# Autodesk Inventor assembly: Electronics V2
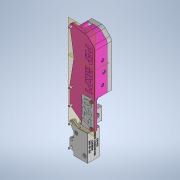
[picture p0: Inventor's stored thumbnail of the model, 180x180]
Saved by Autodesk Inventor 2020.3 (Build 243373010, 373A)
## iProperties
Created: 2019-12-13
Part Number: Electronics V2
Document SubType Name: Assembly
Designer: pepd9
Mass: 362.795 g
Surface Area: 2325.02 cm^2
Volume: 298.236 cm^3
Density: 1.21647 g/cm^3
Author: pepd9
## Documents named in this file (16)
- D:\Designs\MK3PRO P1\ELECTRONICS\Electronics V2.iam
- D:\Designs\MK3PRO P1\COMPONENTS\SHCS_M3_12.ipt
- D:\Designs\MK3PRO P1\COMPONENTS\M3 Nut.ipt
- D:\Designs\MK3PRO P1\ELECTRONICS\LM2596.ipt
- D:\Designs\MK3PRO P1\ELECTRONICS\FAN PS CASE.ipt
- D:\Designs\MK3PRO P1\COMPONENTS\SHCS_M3_8.ipt
- D:\Designs\MK3PRO P1\COMPONENTS\NUT_SQUARE_M3.ipt
- D:\Designs\MK3PRO P1\COMPONENTS\SHCS_M3_10.ipt
- D:\Designs\MK3PRO P1\ELECTRONICS\FAN PS CASE LID.ipt
- D:\Designs\MK3PRO P1\ELECTRONICS\Fan Distribution Case.ipt
- D:\Designs\MK3PRO P1\ELECTRONICS\Double Sided PCB 6x28.iam
- D:\Designs\MK3PRO P1\COMPONENTS\M3 Washer.ipt
- D:\Designs\MK3PRO P1\FRAME\Extruder-Motherboard Cable Clamp.ipt
- D:\Designs\MK3PRO P1\COMPONENTS\SHCS_M3_20.ipt
- D:\Designs\MK3PRO P1\ELECTRONICS\Fan PDP Lid.ipt
- D:\Designs\MK3PRO P1\ELECTRONICS\ID Plate.ipt
## Components (37 placed, 15 different names)
1. LM2596:1 — Mate:18, Mate:19
2. SHCS_M3_8:1 — Mate:19, Mate:24
3. SHCS_M3_8:2 — Mate:18, Mate:23
4. M3 Nut:5 — Mate:24
5. M3 Nut:6 — Mate:23
6. NUT_SQUARE_M3:1
7. SHCS_M3_10:1 — Mate:166
8. SHCS_M3_10:2 — Mate:167
9. SHCS_M3_8:3 — Mate:33, Mate:34
10. FAN PS CASE LID:1 — Mate:33, Mate:34
11. Fan Distribution Case:1 — Mate:35, Angle:10, Mate:36, Mate:37, Mate:42, Mate:44, Mate:47, Mate:56, Mate:57, Mate:58, Mate:59, Angle:11, Angle:12, Mate:64, Mate:65, Mate:66, Mate:67, Mate:72, Mate:73, Mate:74, Mate:75, Angle:15, Angle:16, Mate:76, Mate:77, Mate:84, Angle:17, Mate:86, Angle:18, Mate:138, Mate:139, Mate:140, Mate:142, Mate:147, Flush:1, Mate:149, Flush:2
12. Double Sided PCB 6x28:1 [sub-assembly] — Mate:35, Angle:10, Mate:36, Mate:37
13. Extruder-Motherboard Cable Clamp:2 — Mate:42, Mate:44, Mate:47, Mate:48, Mate:49, Mate:52, Mate:53
14. SHCS_M3_20:2 — Mate:49, Mate:53, Mate:62
15. SHCS_M3_20:4 — Mate:48, Mate:52, Mate:63
16. M3 Nut:7 — Mate:59
17. M3 Nut:8 — Mate:58
18. M3 Nut:9 — Mate:57, Mate:62, Angle:12
19. M3 Nut:10 — Mate:56, Mate:63, Angle:11
20. M3 Nut:11 — Mate:73, Mate:74, Angle:15
21. M3 Nut:12 — Mate:72, Mate:75, Angle:16
22. M3 Washer:2 — Mate:64, Mate:69, Mate:70
23. M3 Washer:3 — Mate:65, Mate:68, Mate:71
24. SHCS_M3_10:4 — Mate:66, Mate:69, Mate:70
25. SHCS_M3_10:5 — Mate:67, Mate:68, Mate:71
26. SHCS_M3_8:4 — Mate:76, Mate:144, Mate:145
27. SHCS_M3_8:5 — Mate:77, Mate:143, Mate:146
28. SHCS_M3_12:3 — Mate:87, Mate:148, Mate:163
29. SHCS_M3_12:4 — Mate:85
30. NUT_SQUARE_M3:2 — Mate:84, Mate:85, Angle:17
31. NUT_SQUARE_M3:3 — Mate:86, Mate:87, Angle:18
32. SHCS_M3_10:6 — Mate:140, Mate:141
33. M3 Washer:6 — Mate:138, Mate:139, Mate:141
34. ID Plate:1 — Mate:142, Mate:143, Mate:144, Mate:145, Mate:146
35. Fan PDP Lid:1 — Mate:147, Mate:148, Flush:1, Mate:149, Mate:163, Mate:164, Mate:165
36. SHCS_M3_12:7 — Mate:164, Mate:165
37. FAN PS CASE:1 — Mate:166, Mate:167, Flush:2
## Relationships (66: Mate 57, Angle 7, Flush 2)
- Mate:18: LM2596:1 ↔ SHCS_M3_8:2
- Mate:19: LM2596:1 ↔ SHCS_M3_8:1
- Mate:23: SHCS_M3_8:2 ↔ M3 Nut:6
- Mate:24: SHCS_M3_8:1 ↔ M3 Nut:5
- Mate:33: SHCS_M3_8:3 ↔ FAN PS CASE LID:1
- Mate:34: SHCS_M3_8:3 ↔ FAN PS CASE LID:1
- Mate:35: Fan Distribution Case:1 ↔ Double Sided PCB 6x28:1
- Angle:10 (0 deg): Fan Distribution Case:1 ↔ Double Sided PCB 6x28:1
- Mate:36 (-40 mm): Fan Distribution Case:1 ↔ Double Sided PCB 6x28:1
- Mate:37 (0.3 mm): Fan Distribution Case:1 ↔ Double Sided PCB 6x28:1
- Mate:42: Fan Distribution Case:1 ↔ Extruder-Motherboard Cable Clamp:2
- Mate:44: Fan Distribution Case:1 ↔ Extruder-Motherboard Cable Clamp:2
- Mate:47: Fan Distribution Case:1 ↔ Extruder-Motherboard Cable Clamp:2
- Mate:48: Extruder-Motherboard Cable Clamp:2 ↔ SHCS_M3_20:4
- Mate:49: Extruder-Motherboard Cable Clamp:2 ↔ SHCS_M3_20:2
- Mate:52: Extruder-Motherboard Cable Clamp:2 ↔ SHCS_M3_20:4
- Mate:53: Extruder-Motherboard Cable Clamp:2 ↔ SHCS_M3_20:2
- Mate:56: Fan Distribution Case:1 ↔ M3 Nut:10
- Mate:57: Fan Distribution Case:1 ↔ M3 Nut:9
- Mate:58: Fan Distribution Case:1 ↔ M3 Nut:8
- Mate:59: Fan Distribution Case:1 ↔ M3 Nut:7
- Mate:62: SHCS_M3_20:2 ↔ M3 Nut:9
- Mate:63: SHCS_M3_20:4 ↔ M3 Nut:10
- Angle:11 (0 deg): Fan Distribution Case:1 ↔ M3 Nut:10
- Angle:12 (0 deg): Fan Distribution Case:1 ↔ M3 Nut:9
- Mate:64: Fan Distribution Case:1 ↔ M3 Washer:2
- Mate:65: Fan Distribution Case:1 ↔ M3 Washer:3
- Mate:66: Fan Distribution Case:1 ↔ SHCS_M3_10:4
- Mate:67: Fan Distribution Case:1 ↔ SHCS_M3_10:5
- Mate:68: M3 Washer:3 ↔ SHCS_M3_10:5
- Mate:69: M3 Washer:2 ↔ SHCS_M3_10:4
- Mate:70: M3 Washer:2 ↔ SHCS_M3_10:4
- Mate:71: M3 Washer:3 ↔ SHCS_M3_10:5
- Mate:72: Fan Distribution Case:1 ↔ M3 Nut:12
- Mate:73: Fan Distribution Case:1 ↔ M3 Nut:11
- Mate:74: Fan Distribution Case:1 ↔ M3 Nut:11
- Mate:75: Fan Distribution Case:1 ↔ M3 Nut:12
- Angle:15 (0 deg): Fan Distribution Case:1 ↔ M3 Nut:11
- Angle:16 (0 deg): Fan Distribution Case:1 ↔ M3 Nut:12
- Mate:76: Fan Distribution Case:1 ↔ SHCS_M3_8:4
- Mate:77: Fan Distribution Case:1 ↔ SHCS_M3_8:5
- Mate:84: Fan Distribution Case:1 ↔ NUT_SQUARE_M3:2
- Mate:85: SHCS_M3_12:4 ↔ NUT_SQUARE_M3:2
- Angle:17 (0 deg): Fan Distribution Case:1 ↔ NUT_SQUARE_M3:2
- Mate:86: Fan Distribution Case:1 ↔ NUT_SQUARE_M3:3
- Mate:87: SHCS_M3_12:3 ↔ NUT_SQUARE_M3:3
- Angle:18 (0 deg): Fan Distribution Case:1 ↔ NUT_SQUARE_M3:3
- Mate:138: Fan Distribution Case:1 ↔ M3 Washer:6
- Mate:139: Fan Distribution Case:1 ↔ M3 Washer:6
- Mate:140: Fan Distribution Case:1 ↔ SHCS_M3_10:6
- Mate:141: SHCS_M3_10:6 ↔ M3 Washer:6
- Mate:142: Fan Distribution Case:1 ↔ ID Plate:1
- Mate:143: SHCS_M3_8:5 ↔ ID Plate:1
- Mate:144: SHCS_M3_8:4 ↔ ID Plate:1
- Mate:145: SHCS_M3_8:4 ↔ ID Plate:1
- Mate:146: SHCS_M3_8:5 ↔ ID Plate:1
- Mate:147: Fan Distribution Case:1 ↔ Fan PDP Lid:1
- Mate:148: SHCS_M3_12:3 ↔ Fan PDP Lid:1
- Flush:1: Fan Distribution Case:1 ↔ Fan PDP Lid:1
- Mate:149: Fan Distribution Case:1 ↔ Fan PDP Lid:1
- Mate:163: SHCS_M3_12:3 ↔ Fan PDP Lid:1
- Mate:164: Fan PDP Lid:1 ↔ SHCS_M3_12:7
- Mate:165: Fan PDP Lid:1 ↔ SHCS_M3_12:7
- Mate:166: SHCS_M3_10:1 ↔ FAN PS CASE:1
- Mate:167: SHCS_M3_10:2 ↔ FAN PS CASE:1
- Flush:2: Fan Distribution Case:1 ↔ FAN PS CASE:1
